# Autodesk Inventor assembly: CoolingModule
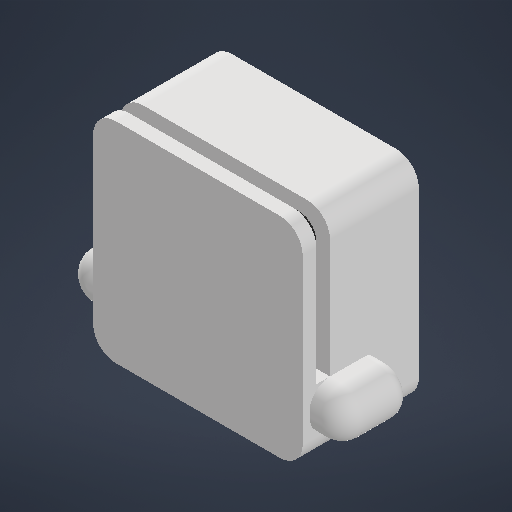
[picture p0: Inventor's stored thumbnail of the model, 512x512]
Saved by Autodesk Inventor 2025 (Build 290162000, 162)
## iProperties
Created: 2024-04-29
Part Number: CoolingModule
Document SubType Name: Assembly
Designer: techn
Author: techn
## Documents named in this file (4)
- C:\Users\techn\OneDrive\devMaxTrauma\3DModel\CoolingModule\CoolingModule.iam
- C:\Users\techn\OneDrive\devMaxTrauma\3DModel\CoolingModule\FANHOLDER.ipt
- C:\Users\techn\OneDrive\devMaxTrauma\3DModel\CoolingModule\40mm-dc-fan-1.snapshot.7\40x40x10 DC Fan\40x40x10 DC Fan.ipt
- C:\Users\techn\OneDrive\devMaxTrauma\3DModel\CoolingModule\FANCATCHER.ipt
## Components (3 placed, 3 different names)
1. FANHOLDER:1 — Rigid:1, Rigid:2
2. 40x40x10 DC Fan:1 — Rigid:1
3. FANCATCHER:1 — Rigid:2
## Relationships (2: WeldJoint 2)
- Rigid:1 [WeldJoint]: FANHOLDER:1 ↔ 40x40x10 DC Fan:1
- Rigid:2 [WeldJoint]: FANHOLDER:1 ↔ FANCATCHER:1
